# Autodesk Inventor assembly: FemaleHeaderPin_1x2
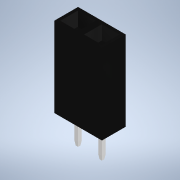
[picture p0: Inventor's stored thumbnail of the model, 180x180]
Saved by Autodesk Inventor 2020 (Build 240168000, 168)
## iProperties
Created: 2020-01-02
Part Number: FemaleHeaderPin_1x2
Document SubType Name: Assembly
Designer: ermoz
Author: ermoz
## Documents named in this file (2)
- D:\Moje Wyczyny\Liceum\VLOat INTvators\Moje projekty\Processor Project (kontynuacja)\Drugie podejście\Electric Elements\FemaleHeaderPin_1x2.iam
- D:\Moje Wyczyny\Liceum\VLOat INTvators\Moje projekty\Processor Project (kontynuacja)\Drugie podejście\Electric Elements\FemaleHederPin.ipt
## Components (2 placed, 1 different names)
1. FemaleHederPin:1 — Mate:1, Flush:1, Flush:7
2. FemaleHederPin:2 — Mate:1, Flush:1, Flush:7
## Relationships (3: Flush 2, Mate 1)
- Mate:1: FemaleHederPin:1 ↔ FemaleHederPin:2
- Flush:1: FemaleHederPin:1 ↔ FemaleHederPin:2
- Flush:7: FemaleHederPin:1 ↔ FemaleHederPin:2
